# Autodesk Inventor assembly: large ball knocker right_MIR
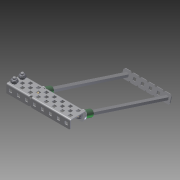
[picture p0: Inventor's stored thumbnail of the model, 180x180]
Saved by Autodesk Inventor 2014 SP1 (Build 180222100, 222)
## iProperties
Created: 2014-03-20
Part Number: large ball knocker right_MIR
Document SubType Name: Assembly
Designer: Ryan
Author: Ryan
## Documents named in this file (8)
- C:\Users\Ryan\Desktop\sw\toss up 5th A bot\tower\large ball knocker right_MIR.iam
- C:\Users\Ryan\Desktop\sw\toss up 5th A bot\tower\large ball knocker metal_MIR.iam
- C:\Users\Ryan\Desktop\sw\lib\Aperture VEX CAD Library\Spacers\SPACER-0500-0125.ipt
- C:\Users\Ryan\Desktop\sw\lib\Super Sonic Sparks VEX CAD Library\Other Parts\(Flexible) Rubber Link.ipt
- C:\Users\Ryan\Desktop\sw\lib\Aperture VEX CAD Library\Hardware\8-32\8-32 nylock.ipt
- C:\Users\Ryan\Desktop\sw\lib\Aperture VEX CAD Library\Standoffs\BEAM-5000.ipt
- C:\Users\Ryan\Desktop\sw\lib\Aperture VEX CAD Library\Hardware\8-32\8-32_.375.ipt
- C:\Users\Ryan\Desktop\sw\lib\Aperture VEX CAD Library\Metal\Custom 1 bar\6.ipt
## Components (16 placed, 7 different names)
1. large ball knocker metal_MIR:1 [sub-assembly] — Mate:2, Mate:1, Mate:3, Mate:6, Mate:5, Mate:4, Mate:11, Mate:14, Mate:20, Mate:19, Mate:18, Mate:23, Mate:22, Mate:21, Mate:25
2. SPACER-0500-0125:1 — Mate:2, Mate:1, Mate:3, Mate:10, Mate:9
3. SPACER-0500-0125:2 — Mate:6, Mate:5, Mate:4, Mate:8, Mate:7
4. (Flexible) Rubber Link:1 — Mate:8, Mate:7, Mate:13, Mate:17, Mate:15
5. (Flexible) Rubber Link:2 — Mate:10, Mate:9, Mate:12, Mate:16
6. 8-32 nylock:1 — Mate:12, Mate:11
7. 8-32 nylock:2 — Mate:14, Mate:13
8. BEAM-5000:1 — Mate:16, Flush:1, Mate:29, Mate:28, Mate:27, Mate:31
9. BEAM-5000:2 — Mate:17, Flush:1, Mate:15, Mate:30, Mate:33
10. 8-32_.375:1 — Mate:20, Mate:19, Mate:18, Mate:26
11. 8-32_.375:2 — Mate:23, Mate:22, Mate:21, Mate:24
12. 8-32 nylock:3 — Mate:25, Mate:24, Flush:2
13. 8-32 nylock:4 — Mate:26, Flush:2
14. 6:1 — Mate:30, Mate:29, Mate:28, Mate:27, Mate:32, Mate:34
15. 8-32_.375:3 — Mate:32, Mate:31
16. 8-32_.375:4 — Mate:34, Mate:33
## Relationships (36: Mate 34, Flush 2)
- Mate:2 (2.3114 mm): large ball knocker metal_MIR:1 ↔ SPACER-0500-0125:1
- Mate:1: large ball knocker metal_MIR:1 ↔ SPACER-0500-0125:1
- Mate:3 (2.3114 mm): large ball knocker metal_MIR:1 ↔ SPACER-0500-0125:1
- Mate:6 (2.3114 mm): large ball knocker metal_MIR:1 ↔ SPACER-0500-0125:2
- Mate:5 (2.3114 mm): large ball knocker metal_MIR:1 ↔ SPACER-0500-0125:2
- Mate:4: large ball knocker metal_MIR:1 ↔ SPACER-0500-0125:2
- Mate:8: SPACER-0500-0125:2 ↔ (Flexible) Rubber Link:1
- Mate:7: SPACER-0500-0125:2 ↔ (Flexible) Rubber Link:1
- Mate:10: SPACER-0500-0125:1 ↔ (Flexible) Rubber Link:2
- Mate:9: SPACER-0500-0125:1 ↔ (Flexible) Rubber Link:2
- Mate:12: (Flexible) Rubber Link:2 ↔ 8-32 nylock:1
- Mate:11: large ball knocker metal_MIR:1 ↔ 8-32 nylock:1
- Mate:14: large ball knocker metal_MIR:1 ↔ 8-32 nylock:2
- Mate:13: (Flexible) Rubber Link:1 ↔ 8-32 nylock:2
- Mate:16: (Flexible) Rubber Link:2 ↔ BEAM-5000:1
- Mate:17: (Flexible) Rubber Link:1 ↔ BEAM-5000:2
- Flush:1: BEAM-5000:1 ↔ BEAM-5000:2
- Mate:15: (Flexible) Rubber Link:1 ↔ BEAM-5000:2
- Mate:20 (2.3114 mm): large ball knocker metal_MIR:1 ↔ 8-32_.375:1
- Mate:19 (2.3114 mm): large ball knocker metal_MIR:1 ↔ 8-32_.375:1
- Mate:18: large ball knocker metal_MIR:1 ↔ 8-32_.375:1
- Mate:23: large ball knocker metal_MIR:1 ↔ 8-32_.375:2
- Mate:22 (2.3114 mm): large ball knocker metal_MIR:1 ↔ 8-32_.375:2
- Mate:21 (2.3114 mm): large ball knocker metal_MIR:1 ↔ 8-32_.375:2
- Mate:25 (1.1684 mm): large ball knocker metal_MIR:1 ↔ 8-32 nylock:3
- Mate:24: 8-32_.375:2 ↔ 8-32 nylock:3
- Mate:26: 8-32_.375:1 ↔ 8-32 nylock:4
- Flush:2: 8-32 nylock:3 ↔ 8-32 nylock:4
- Mate:30 (2.3114 mm): BEAM-5000:2 ↔ 6:1
- Mate:29 (2.3114 mm): BEAM-5000:1 ↔ 6:1
- Mate:28 (2.3114 mm): BEAM-5000:1 ↔ 6:1
- Mate:27: BEAM-5000:1 ↔ 6:1
- Mate:32: 6:1 ↔ 8-32_.375:3
- Mate:31: BEAM-5000:1 ↔ 8-32_.375:3
- Mate:34: 6:1 ↔ 8-32_.375:4
- Mate:33: BEAM-5000:2 ↔ 8-32_.375:4
